# Autodesk Inventor assembly: kick
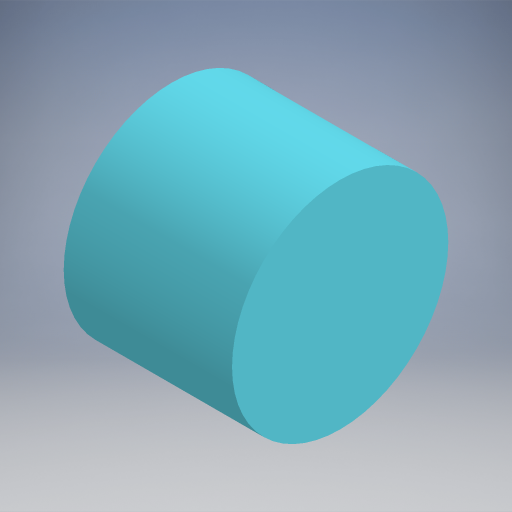
[picture p0: Inventor's stored thumbnail of the model, 512x512]
Saved by Autodesk Inventor 2023 (Build 270158000, 158)
## iProperties
Created: 2025-03-27
Part Number: kick
Document SubType Name: Assembly
Designer: Ivan
Author: Ivan
## Documents named in this file (3)
- C:\!projects\DASH-\3D\Dash-V1\Solenoid\kick.iam
- C:\Users\Ivan\Documents\Inventor\Content Center Files\R2023\ru-RU\ANSI B18.2.4.2M\ANSI B18.2.4.2M - M5x0,8 - 8.ipt
- C:\!projects\DASH-\3D\Dash-V1\Solenoid\kicker.ipt
## Components (2 placed, 2 different names)
1. ANSI B18.2.4.2M M5x0,8:1 — Совмещение:1, Заподлицо:1, Угол:1
2. kicker:1 — Заподлицо:2, Заподлицо:3
## Relationships (5: Flush 3, Mate 1, Angle 1)
- Совмещение:1 [Mate]: ANSI B18.2.4.2M M5x0,8:1
- Заподлицо:1 [Flush]: ANSI B18.2.4.2M M5x0,8:1
- Заподлицо:2 [Flush]: kicker:1
- Заподлицо:3 [Flush]: kicker:1
- Угол:1 [Angle] (0 deg): ANSI B18.2.4.2M M5x0,8:1
